# Autodesk Inventor assembly: Assembly1
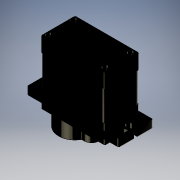
[picture p0: Inventor's stored thumbnail of the model, 180x180]
Saved by Autodesk Inventor 2019 (Build 230136000, 136)
## iProperties
Created: 2021-01-14
Part Number: Assembly1
Document SubType Name: Assembly
Designer: CS
Author: CS
## Documents named in this file (18)
- C:\Users\caspe\OneDrive\Documenten\Inventor\servo\inventor files\Assembly1.iam
- C:\Users\caspe\OneDrive\Documenten\Inventor\servo\inventor files\servo midden.ipt
- C:\Users\caspe\OneDrive\Documenten\Inventor\servo\inventor files\sevo boven.ipt
- C:\Users\caspe\OneDrive\Documenten\Inventor\servo\inventor files\sevo onder.ipt
- C:\Users\caspe\OneDrive\Documenten\Inventor\servo\inventor files\motor.ipt
- C:\Users\caspe\OneDrive\Documenten\Inventor\servo\inventor files\asje klein.ipt
- C:\Users\caspe\OneDrive\Documenten\Inventor\servo\inventor files\asje groot.ipt
- C:\Users\caspe\OneDrive\Documenten\Inventor\servo\Assembly1\Design Accelerator\Spur Gears1.iam
- C:\Users\caspe\OneDrive\Documenten\Inventor\servo\Assembly1\Design Accelerator\Spur Gears2.iam
- C:\Users\caspe\OneDrive\Documenten\Inventor\servo\Assembly1\Design Accelerator\Spur Gears3.iam
- C:\Users\caspe\OneDrive\Documenten\Inventor\servo\Assembly1\Design Accelerator\Spur Gears4.iam
- C:\Users\caspe\OneDrive\Documenten\Inventor\servo\inventor files\sticker.ipt
- C:\Users\caspe\OneDrive\Documenten\Inventor\servo\inventor files\screw.ipt
- C:\Users\caspe\OneDrive\Documenten\Inventor\servo\Assembly servo inside.ipt
- C:\Users\caspe\OneDrive\Documenten\Inventor\servo\Assembly servo outside.ipt
- C:\Users\caspe\OneDrive\Afbeeldingen\white bumps.jpg
- C:\Users\caspe\OneDrive\Afbeeldingen\aluminum_texture1639.jpg
- C:\Users\caspe\Downloads\20210119_143510.jpg
## Components (18 placed, 11 different names)
1. servo midden:1 — Insert:1, Angle:1, Insert:3, Insert:4, Insert:5, Insert:6, Insert:7, Mate:5, Mate:9, Mate:18, Mate:19
2. motor:1 — Insert:1, Angle:1, Mate:1, Angle:2, Flush:1, Mate:2, Mate:3
3. sevo boven:1 — Insert:5, Insert:6
4. sevo onder:1 — Insert:3, Insert:4, Mate:21, Insert:8, Insert:9, Insert:10, Insert:11
5. asje klein:1 — Insert:7, Mate:4, Mate:6, Mate:12, Mate:14
6. asje groot:1 — Mate:1, Angle:2, Flush:1, Mate:8, Mate:10, Mate:16
7. Spur Gears:1 [sub-assembly] — Mate:2, Mate:3, Mate:4, Mate:5, Mate:7
8. Spur Gears:2 [sub-assembly] — Mate:6, Mate:7, Mate:8, Mate:9, Mate:11, Mate:13
9. Spur Gears:3 [sub-assembly] — Mate:10, Mate:11, Mate:12, Mate:13, Mate:15, Mate:17
10. Spur Gears:4 [sub-assembly] — Mate:14, Mate:15, Mate:16, Mate:17
11. sticker:1 — Mate:18, Flush:2, Flush:3, Mate:21
12. sticker:2 — Mate:19, Mate:20, Flush:3
13. screw:1 — Insert:11
14. screw:2 — Insert:10
15. screw:3 — Insert:9
16. screw:4 — Insert:8
17. Assembly servo inside:1
18. Assembly servo outside:1
## Relationships (36: Mate 21, Insert 10, Flush 3, Angle 2)
- Insert:1: servo midden:1 ↔ motor:1
- Angle:1 (0 deg): servo midden:1 ↔ motor:1
- Insert:3: servo midden:1 ↔ sevo onder:1
- Insert:4: servo midden:1 ↔ sevo onder:1
- Insert:5: servo midden:1 ↔ sevo boven:1
- Insert:6: servo midden:1 ↔ sevo boven:1
- Insert:7: servo midden:1 ↔ asje klein:1
- Mate:1: motor:1 ↔ asje groot:1
- Angle:2 (90 deg): motor:1 ↔ asje groot:1
- Flush:1: motor:1 ↔ asje groot:1
- Mate:2: motor:1 ↔ Spur Gears:1
- Mate:3: motor:1 ↔ Spur Gears:1
- Mate:4: asje klein:1 ↔ Spur Gears:1
- Mate:5: servo midden:1 ↔ Spur Gears:1
- Mate:6: asje klein:1 ↔ Spur Gears:2
- Mate:7: Spur Gears:1 ↔ Spur Gears:2
- Mate:8: asje groot:1 ↔ Spur Gears:2
- Mate:9: servo midden:1 ↔ Spur Gears:2
- Mate:10: asje groot:1 ↔ Spur Gears:3
- Mate:11: Spur Gears:2 ↔ Spur Gears:3
- Mate:12: asje klein:1 ↔ Spur Gears:3
- Mate:13: Spur Gears:2 ↔ Spur Gears:3
- Mate:14: asje klein:1 ↔ Spur Gears:4
- Mate:15: Spur Gears:3 ↔ Spur Gears:4
- Mate:16: asje groot:1 ↔ Spur Gears:4
- Mate:17: Spur Gears:3 ↔ Spur Gears:4
- Mate:18: servo midden:1 ↔ sticker:1
- Flush:2: sticker:1
- Mate:19: servo midden:1 ↔ sticker:2
- Mate:20: sticker:2
- Flush:3: sticker:1 ↔ sticker:2
- Mate:21 (0.25 mm): sevo onder:1 ↔ sticker:1
- Insert:8: sevo onder:1 ↔ screw:4
- Insert:9: sevo onder:1 ↔ screw:3
- Insert:10: sevo onder:1 ↔ screw:2
- Insert:11: sevo onder:1 ↔ screw:1
